# Autodesk Inventor assembly: Assembly1
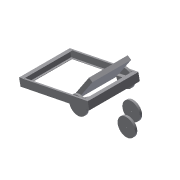
[picture p0: Inventor's stored thumbnail of the model, 180x180]
Saved by Autodesk Inventor 2015 (Build 190159000, 159)
## iProperties
Created: 2015-03-05
Part Number: Assembly1
Document SubType Name: Assembly
Designer: Kyle
Author: Kyle
## Documents named in this file (6)
- C:\Users\Kyle\Documents\Inventor\ReDesign\Assembly1.iam
- C:\Users\Kyle\Documents\Inventor\ReDesign\FrameFandB.ipt
- C:\Users\Kyle\Documents\Inventor\ReDesign\FrameSide.ipt
- C:\Users\Kyle\Documents\Inventor\ReDesign\ControlBoard.ipt
- C:\Users\Kyle\Documents\Inventor\ReDesign\Toughbox+Nano+All+Shafts+v2.iam
- C:\Users\Kyle\Documents\Inventor\ReDesign\Wheel.ipt
## Components (11 placed, 5 different names)
1. FrameFandB:1 — Mate:5, Mate:6, Mate:7, Angle:1, Mate:22
2. FrameFandB:2 — Mate:1, Mate:2, Mate:3, Mate:4, Flush:1, Flush:2
3. FrameSide:1 — Mate:1, Mate:2, Mate:5, Mate:6, Flush:1, Flush:7
4. FrameSide:2 — Mate:3, Mate:4, Mate:7, Flush:2, Mate:19, Flush:6
5. ControlBoard:1 — Mate:19, Angle:1, Mate:20, Mate:21, Mate:22
6. Toughbox+Nano+All+Shafts+v2:1 [sub-assembly] — Mate:18, Flush:5, Mate:20
7. Toughbox+Nano+All+Shafts+v2:2 [sub-assembly] — Mate:17, Flush:4, Mate:21
8. Wheel:1
9. Wheel:2 — Mate:17, Flush:4, Flush:6
10. Wheel:3 — Mate:18, Flush:5, Flush:7
11. Wheel:4
## Relationships (20: Mate 13, Flush 6, Angle 1)
- Mate:1: FrameFandB:2 ↔ FrameSide:1
- Mate:2: FrameFandB:2 ↔ FrameSide:1
- Mate:3: FrameFandB:2 ↔ FrameSide:2
- Mate:4: FrameFandB:2 ↔ FrameSide:2
- Mate:5: FrameFandB:1 ↔ FrameSide:1
- Mate:6: FrameFandB:1 ↔ FrameSide:1
- Mate:7: FrameFandB:1 ↔ FrameSide:2
- Flush:1: FrameFandB:2 ↔ FrameSide:1
- Flush:2: FrameFandB:2 ↔ FrameSide:2
- Mate:17: Toughbox+Nano+All+Shafts+v2:2 ↔ Wheel:2
- Flush:4: Toughbox+Nano+All+Shafts+v2:2 ↔ Wheel:2
- Mate:18: Toughbox+Nano+All+Shafts+v2:1 ↔ Wheel:3
- Flush:5: Toughbox+Nano+All+Shafts+v2:1 ↔ Wheel:3
- Mate:19 (67.564 mm): FrameSide:2 ↔ ControlBoard:1
- Angle:1 (135 deg): FrameFandB:1 ↔ ControlBoard:1
- Mate:20: ControlBoard:1 ↔ Toughbox+Nano+All+Shafts+v2:1
- Mate:21: ControlBoard:1 ↔ Toughbox+Nano+All+Shafts+v2:2
- Flush:6 (25.4 mm): FrameSide:2 ↔ Wheel:2
- Flush:7 (25.4 mm): FrameSide:1 ↔ Wheel:3
- Mate:22 (203.2 mm): FrameFandB:1 ↔ ControlBoard:1
